# Autodesk Inventor assembly: SCBRJ12-15
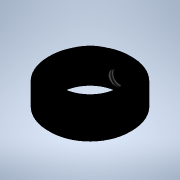
[picture p0: Inventor's stored thumbnail of the model, 180x180]
Saved by Autodesk Inventor 2021 (Build 250183000, 183)
## iProperties
Category: PARTsolutions
Company: MISUMI
Created: 2025-04-04
Part Number: SCBRJ12-15
Catalog Web Link: www.cadenas.de
Description: SCBRJ, PSCBRJ, SSCBRJ, SCSRAJ, SCSRAWJ, SCBSJ, PSCBSJ, SSCBSJ-Set Collars - For Bearing Fixing - (For Space Saving) - Set Screw Compact Type
Vendor: MISUMI
Document SubType Name: Assembly
Designer: psAdmin
Manufacturer: MISUMI
Mass: 1.08635 g
Surface Area: 11.4493 cm^2
Volume: 1.08635 cm^3
Density: 1 g/cm^3
Title: SCBRJ12-15
Author: Cadenas PARTsolutions
Comments: Set Collars - For Bearing Fixing - (For Space Saving) - Set Screw Compact Type
PSOL_IDENT_0: {$CADENAS_DATA/23d-libs/misumi/metric/03_set_collars/scbrj_asmtab.prj},245 {VTYP=3D},{STYP=ASSTAB},{
PSOL_IDENT_1: NB=SCBRJ12-15},{LINA=SCBRJ12-15},{NN=SCBRJ, PSCBRJ, SSCBRJ, SCSRAJ, SCSRAWJ, SCBSJ, PSCBSJ, SSCBSJ},
PSOL_IDENT_2: {DATE=02.11.2021 00:56:17},{GEOMDATE=19.10.2021 09:37:10},{VERSION=},{LINEID=70},{WBVAR=TS,MAT,ST,DS
PSOL_IDENT_3: S},{WBNUMERIC=DSS}  {NB=SCBRJ12-15},{LINA=SCBRJ12-15},{KT=DUMMY},{PN=SCBRJ12-15},{D=12},{TYPE=SCBRJ}
PSOL_IDENT_4: ,{TS=SN},{MAT=1045},{MATA='1045','1045 Carbon Steel','304','SUS304 Equivalent','2017','2017 Aluminum
PSOL_IDENT_5: Alloy'},{ST=Black Oxide},{AC=Set Screws 2 Pcs.},{DSS=15},{DS1=15,16,18},{AB=6701ZZ(18)-6801ZZ(21)},
PSOL_IDENT_6: {B=7.5},{B11=7.5},{B1=0},{B12=10},{D1=19},{M=M4x3},{THMD=4},{THDMIN=3.242},{BB=6},{ST0='Black Oxide'
PSOL_IDENT_7: ,'Black Oxide','Electroless Nickel Plating','Electroless Nickel Plating'},{C=0.5},{L=3},{TS1='SN','S
PSOL_IDENT_8: hort Nose','LN','Long Nose'},{PPATH=scbrj/scbrj_templ.prj},{LTHREAD=3},{TIFF=1}
NB: SCBRJ12-15
NN: SCBRJ, PSCBRJ, SSCBRJ, SCSRAJ, SCSRAWJ, SCBSJ, PSCBSJ, SSCBSJ
NT: Set Collars - For Bearing Fixing - (For Space Saving) - Set Screw Compact Type
NBSYN: $PN.
LINA: SCBRJ12-15
CATALOG: Misumi
PN: SCBRJ12-15
D: 12
TS: Short Nose
MAT: 1045 Carbon Steel
ST: Black Oxide
AC: Set Screws 2 Pcs.
DSS: 15
AB: 6701ZZ(18)-6801ZZ(21)
B: 7.5
B1: 0
D1: 19
M: M4x3
BB: 6
SUPPLIER: MISUMI
ARTICLENO: SCBRJ12-15
BOMINFO: SCBRJ12-15
CREATOR: CADENAS GmbH
## Documents named in this file (3)
- e:\temp\worker_COMMON_84\temp\tmp_10120_258_eS1mG\format_0\SCBRJ12-15.iam
- e:\temp\worker_COMMON_84\temp\tmp_10120_258_eS1mG\format_0\SCBRJ12-15_b.ipt
- e:\temp\worker_COMMON_84\temp\tmp_10120_258_eS1mG\format_0\Hexagon socket set screw with flat point DIN 913 - M4x3.ipt
## Components (3 placed, 2 different names)
1. SCBRJ12-15_b:1 — body_set_v_Z@1 <-> IP1_Z@2, body_set_h_Z@1 <-> IP1_Z@3
2. Hexagon socket set screw with flat point DIN 913 - M4x3:1 — body_set_v_Z@1 <-> IP1_Z@2
3. Hexagon socket set screw with flat point DIN 913 - M4x3:2 — body_set_h_Z@1 <-> IP1_Z@3
## Relationships (2: Mate 2)
- body_set_v_Z@1 <-> IP1_Z@2 [Mate]: SCBRJ12-15_b:1 ↔ Hexagon socket set screw with flat point DIN 913 - M4x3:1
- body_set_h_Z@1 <-> IP1_Z@3 [Mate]: SCBRJ12-15_b:1 ↔ Hexagon socket set screw with flat point DIN 913 - M4x3:2
